# Autodesk Inventor assembly: robot
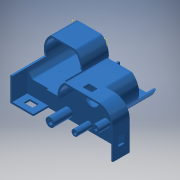
[picture p0: Inventor's stored thumbnail of the model, 180x180]
Saved by Autodesk Inventor 2017 (Build 210142000, 142)
## iProperties
Created: 2016-09-07
Part Number: robot
Document SubType Name: Assembly
Designer: Paulo Loma
Author: Paulo Loma
## Documents named in this file (25)
- C:\Users\zurits\Google Drive\IEA_Robotics\IEA_uRobots_v1\mechanics\robot.iam
- C:\Users\zurits\Google Drive\IEA_Robotics\IEA_uRobots_v1\mechanics\rueda.ipt
- C:\Users\zurits\Google Drive\IEA_Robotics\IEA_uRobots_v1\mechanics\motor.ipt
- C:\Users\zurits\Google Drive\IEA_Robotics\IEA_uRobots_v1\mechanics\encoder.ipt
- C:\Users\zurits\Google Drive\IEA_Robotics\IEA_uRobots_v1\mechanics\opto.ipt
- C:\Users\zurits\Google Drive\IEA_Robotics\IEA_uRobots_v1\mechanics\bateria.ipt
- C:\Users\zurits\Google Drive\IEA_Robotics\IEA_uRobots_v1\mechanics\frame2.ipt
- C:\Users\zurits\Google Drive\IEA_Robotics\IEA_uRobots_v1\mechanics\spherical caster wheel.ipt
- C:\Users\zurits\Google Drive\IEA_Robotics\IEA_uRobots_v1\mechanics\frame3.ipt
- C:\Users\zurits\Google Drive\IEA_Robotics\IEA_uRobots_v1\mechanics\frame4.ipt
- C:\Users\zurits\Google Drive\IEA_Robotics\IEA_uRobots_v1\mechanics\frame5.ipt
- C:\Users\zurits\Google Drive\IEA_Robotics\IEA_uRobots_v1\mechanics\robot\Design Accelerator\Spur Gears9.iam
- C:\Users\zurits\Google Drive\IEA_Robotics\IEA_uRobots_v1\mechanics\robot\Design Accelerator\Spur Gears10.iam
- C:\Users\zurits\Google Drive\IEA_Robotics\IEA_uRobots_v1\mechanics\robot\Design Accelerator\Spur Gears11.iam
- C:\Users\zurits\Google Drive\IEA_Robotics\IEA_uRobots_v1\mechanics\robot\Design Accelerator\Spur Gears12.iam
- C:\Users\zurits\Google Drive\IEA_Robotics\IEA_uRobots_v1\mechanics\rueda_MIR4_MIR.ipt
- C:\Users\zurits\Google Drive\IEA_Robotics\IEA_uRobots_v1\mechanics\motor_MIR4_MIR.ipt
- C:\Users\zurits\Google Drive\IEA_Robotics\IEA_uRobots_v1\mechanics\encoder_MIR4_MIR.ipt
- C:\Users\zurits\Google Drive\IEA_Robotics\IEA_uRobots_v1\mechanics\opto_MIR4_MIR.ipt
- C:\Users\zurits\Google Drive\IEA_Robotics\IEA_uRobots_v1\mechanics\robot\Design Accelerator\Spur Gears9_MIR1_MIR2.iam
- C:\Users\zurits\Google Drive\IEA_Robotics\IEA_uRobots_v1\mechanics\robot\Design Accelerator\Spur Gears10_MIR1_MIR2.iam
- C:\Users\zurits\Google Drive\IEA_Robotics\IEA_uRobots_v1\mechanics\robot\Design Accelerator\Spur Gears11_MIR1_MIR2.iam
- C:\Users\zurits\Google Drive\IEA_Robotics\IEA_uRobots_v1\mechanics\robot\Design Accelerator\Spur Gears12_MIR1_MIR2.iam
- C:\Users\zurits\Google Drive\IEA_Robotics\IEA_uRobots_v1\mechanics\frame1.ipt
- C:\Users\zurits\Google Drive\IEA_Robotics\IEA_uRobots_v1\mechanics\frame1b.ipt
## Components (29 placed, 21 different names)
1. rueda:1 — Mate:42, Mate:43, Mate:64
2. motor:1 — Flush:25, Mate:21, Mate:22, Mate:28, Flush:24, Flush:42, Flush:43, Flush:44, Flush:45
3. encoder:1 — Mate:28, Flush:24
4. opto:1 — Flush:25
5. bateria:1 — Mate:19, Flush:13, Flush:16
6. bateria:2 — Mate:19, Flush:13, Flush:16, Flush:17
7. frame2:1 — Flush:17
8. spherical caster wheel:1
9. frame3:1 — Flush:19, Flush:20
10. frame4:1 — Flush:19
11. frame5:1 — Flush:20
12. Spur Gears:2 [sub-assembly] — Mate:36, Mate:37, Tangent:2, Mate:40
13. Spur Gears:3 [sub-assembly] — Mate:36, Mate:37, Tangent:1, Flush:32
14. Spur Gears:4 [sub-assembly] — Mate:21, Mate:22, Tangent:1, Flush:32
15. Spur Gears:5 [sub-assembly] — Tangent:3, Mate:41, Mate:42, Mate:43
16. Spur Gears:6 [sub-assembly] — Tangent:3, Mate:41
17. Spur Gears:7 [sub-assembly] — Tangent:2, Mate:40
18. rueda_MIR4_MIR:1 — Mate:58, Mate:59, Mate:64
19. motor_MIR4_MIR:1 — Mate:53, Flush:39, Flush:40, Mate:56, Mate:57, Flush:42, Flush:43, Flush:44, Flush:46
20. encoder_MIR4_MIR:1 — Mate:53, Flush:39
21. opto_MIR4_MIR:1 — Flush:40
22. Spur Gears9_MIR1_MIR2:1 [sub-assembly] — Mate:54, Mate:55, Tangent:9, Mate:63
23. Spur Gears10_MIR1_MIR2:1 [sub-assembly] — Mate:54, Mate:55, Tangent:7, Flush:41
24. Spur Gears11_MIR1_MIR2:1 [sub-assembly] — Mate:56, Mate:57, Tangent:7, Flush:41
25. Spur Gears12_MIR1_MIR2:1 [sub-assembly] — Mate:58, Mate:59, Tangent:8, Mate:60
26. Spur Gears9_MIR1_MIR2:2 [sub-assembly] — Tangent:8, Mate:60, Mate:61, Mate:62
27. Spur Gears10_MIR1_MIR2:2 [sub-assembly] — Mate:61, Mate:62, Tangent:9, Mate:63
28. frame1a:1 — Flush:45, Flush:46, Flush:47, Flush:48
29. frame1b:1 — Flush:47, Flush:48
## Relationships (48: Mate 24, Flush 18, Tangent 6)
- Flush:25: motor:1 ↔ opto:1
- Mate:19: bateria:1 ↔ bateria:2
- Flush:13: bateria:1 ↔ bateria:2
- Flush:16: bateria:1 ↔ bateria:2
- Flush:17: bateria:2 ↔ frame2:1
- Flush:19: frame3:1 ↔ frame4:1
- Flush:20: frame3:1 ↔ frame5:1
- Mate:21: motor:1 ↔ Spur Gears:4
- Mate:22: motor:1 ↔ Spur Gears:4
- Mate:28: motor:1 ↔ encoder:1
- Flush:24: motor:1 ↔ encoder:1
- Mate:36: Spur Gears:2 ↔ Spur Gears:3
- Mate:37: Spur Gears:2 ↔ Spur Gears:3
- [Mate]: Spur Gears:6 ↔ Spur Gears:7
- [Mate]: Spur Gears:6 ↔ Spur Gears:7
- Tangent:1: Spur Gears:3 ↔ Spur Gears:4
- Flush:32: Spur Gears:3 ↔ Spur Gears:4
- Tangent:2: Spur Gears:2 ↔ Spur Gears:7
- Mate:40: Spur Gears:2 ↔ Spur Gears:7
- Tangent:3: Spur Gears:5 ↔ Spur Gears:6
- Mate:41: Spur Gears:5 ↔ Spur Gears:6
- Mate:42: rueda:1 ↔ Spur Gears:5
- Mate:43: rueda:1 ↔ Spur Gears:5
- Mate:53: motor_MIR4_MIR:1 ↔ encoder_MIR4_MIR:1
- Flush:39: motor_MIR4_MIR:1 ↔ encoder_MIR4_MIR:1
- Flush:40: motor_MIR4_MIR:1 ↔ opto_MIR4_MIR:1
- Mate:54: Spur Gears9_MIR1_MIR2:1 ↔ Spur Gears10_MIR1_MIR2:1
- Mate:55: Spur Gears9_MIR1_MIR2:1 ↔ Spur Gears10_MIR1_MIR2:1
- Mate:56: motor_MIR4_MIR:1 ↔ Spur Gears11_MIR1_MIR2:1
- Mate:57: motor_MIR4_MIR:1 ↔ Spur Gears11_MIR1_MIR2:1
- Tangent:7: Spur Gears10_MIR1_MIR2:1 ↔ Spur Gears11_MIR1_MIR2:1
- Flush:41: Spur Gears10_MIR1_MIR2:1 ↔ Spur Gears11_MIR1_MIR2:1
- Mate:58: rueda_MIR4_MIR:1 ↔ Spur Gears12_MIR1_MIR2:1
- Mate:59: rueda_MIR4_MIR:1 ↔ Spur Gears12_MIR1_MIR2:1
- Tangent:8: Spur Gears12_MIR1_MIR2:1 ↔ Spur Gears9_MIR1_MIR2:2
- Mate:60: Spur Gears12_MIR1_MIR2:1 ↔ Spur Gears9_MIR1_MIR2:2
- Mate:61: Spur Gears9_MIR1_MIR2:2 ↔ Spur Gears10_MIR1_MIR2:2
- Mate:62: Spur Gears9_MIR1_MIR2:2 ↔ Spur Gears10_MIR1_MIR2:2
- Tangent:9: Spur Gears9_MIR1_MIR2:1 ↔ Spur Gears10_MIR1_MIR2:2
- Mate:63: Spur Gears9_MIR1_MIR2:1 ↔ Spur Gears10_MIR1_MIR2:2
- Flush:42: motor:1 ↔ motor_MIR4_MIR:1
- Mate:64: rueda:1 ↔ rueda_MIR4_MIR:1
- Flush:43: motor:1 ↔ motor_MIR4_MIR:1
- Flush:44: motor:1 ↔ motor_MIR4_MIR:1
- Flush:45: motor:1 ↔ frame1a:1
- Flush:46: motor_MIR4_MIR:1 ↔ frame1a:1
- Flush:47: frame1a:1 ↔ frame1b:1
- Flush:48 (18 mm): frame1a:1 ↔ frame1b:1
## Named parameters: d289_d285 = 0 mm, d290_d286 = 0 mm
